# Autodesk Inventor assembly: LM2_lensholder_on_mount
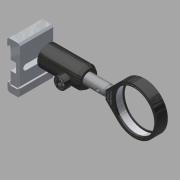
[picture p0: Inventor's stored thumbnail of the model, 180x180]
Saved by Autodesk Inventor 2018 (Build 220112000, 112)
## iProperties
Created: 2018-09-24
Part Number: LM2_lensholder_on_mount
Document SubType Name: Assembly
Designer: Robert Campbell
Author: Robert Campbell
## Documents named in this file (5)
- X:\home\work\Documents\MF_BenchOptics\CAD_files\LM2_lensholder_on_mount.iam
- W:\home\work\Documents\MF_BenchOptics\CAD_files\TR50_M-Solidworks.ipt
- W:\home\work\Documents\MF_BenchOptics\CAD_files\PH50_M-Solidworks.ipt
- W:\home\work\Documents\MF_BenchOptics\CAD_files\XT66C4-Step.ipt
- W:\home\work\Documents\MF_BenchOptics\CAD_files\LMR2_M-Solidworks.ipt
## Components (4 placed, 4 different names)
1. TR50_M-Solidworks:1 — Mate:1, Mate:2, Mate:3, Mate:4, Mate:6
2. PH50_M-Solidworks:1 — Mate:1, Mate:2, Mate:5
3. XT66C4-Step:1 — Mate:5, Mate:6, Angle:1
4. LMR2_M-Solidworks:1 — Mate:3, Mate:4, Angle:1
## Relationships (7: Mate 6, Angle 1)
- Mate:1: TR50_M-Solidworks:1 ↔ PH50_M-Solidworks:1
- Mate:2 (20 mm): TR50_M-Solidworks:1 ↔ PH50_M-Solidworks:1
- Mate:3: TR50_M-Solidworks:1 ↔ LMR2_M-Solidworks:1
- Mate:4: TR50_M-Solidworks:1 ↔ LMR2_M-Solidworks:1
- Mate:5: PH50_M-Solidworks:1 ↔ XT66C4-Step:1
- Mate:6: TR50_M-Solidworks:1 ↔ XT66C4-Step:1
- Angle:1 (0 deg): XT66C4-Step:1 ↔ LMR2_M-Solidworks:1
